# Autodesk Inventor assembly: Marcador
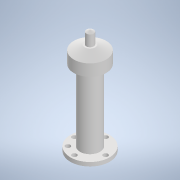
[picture p0: Inventor's stored thumbnail of the model, 180x180]
Saved by Autodesk Inventor 2022 (Build 260153000, 153)
## iProperties
Created: 2022-08-28
Part Number: Marcador
Document SubType Name: Assembly
Designer: Usuario
Author: Usuario
## Documents named in this file (4)
- C:\Users\Usuario\Desktop\Semestre 8\Robotica\Portamarcad\Marcador.iam
- C:\Users\Usuario\Desktop\Semestre 8\Robotica\Portamarcad\Parte superior.ipt
- C:\Users\Usuario\Desktop\Semestre 8\Robotica\Portamarcad\Base.ipt
- C:\Users\Usuario\Desktop\Semestre 8\Robotica\Portamarcad\PuntaMarcador.ipt
## Components (3 placed, 3 different names)
1. Parte superior:1 — Mate:1, Cylindrical:1, Cylindrical:2, Flush:1
2. Base:1 — Cylindrical:2, Flush:1, Mate:2
3. PuntaMarcador:1 — Mate:1, Cylindrical:1
## Relationships (5: Mate 2, CylindricalJoint 2, Flush 1)
- Mate:1: Parte superior:1 ↔ PuntaMarcador:1
- Cylindrical:1: Parte superior:1 ↔ PuntaMarcador:1
- Cylindrical:2: Parte superior:1 ↔ Base:1
- Flush:1 (-4.5 mm): Parte superior:1 ↔ Base:1
- Mate:2: Base:1
